# Autodesk Inventor assembly: ArmFrameWithMotorAndGears
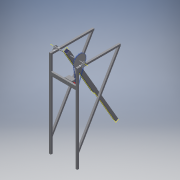
[picture p0: Inventor's stored thumbnail of the model, 180x180]
Saved by Autodesk Inventor 2018.2 (Build 222227000, 227)
## iProperties
Created: 2018-02-07
Part Number: ArmFrameWithMotorAndGears
Document SubType Name: Assembly
Designer: steele
Author: steele
## Documents named in this file (14)
- D:\snobotics\CAD-Development\robSteele\2018-FRC\Arm\ArmFrameWithMotorAndGears.iam
- D:\snobotics\CAD-Development\robSteele\2018-FRC\Arm\armFrame.ipt
- D:\snobotics\CAD-Development\robSteele\2018-FRC\Arm\hexExtrusion.ipt
- D:\snobotics\CAD-Development\robSteele\2018-FRC\Arm\ArmFrameWithMotorAndGears\Design Accelerator\Chain Drive1.iam
- D:\snobotics\CAD-Development\robSteele\2018-FRC\Arm\AM Rev 3209 Motor Mount.ipt
- D:\snobotics\CAD-Development\robSteele\2018-FRC\Arm\BaneBot220GearBox.ipt
- D:\snobotics\CAD-Development\robSteele\2018-FRC\Arm\2inSquareArmTube.ipt
- D:\snobotics\CAD-Development\robSteele\2018-FRC\Arm\1_5inSquareArmTube.ipt
- D:\snobotics\CAD-Development\robSteele\2018-FRC\Arm\30-60-supportBrace.ipt
- D:\snobotics\CAD-Development\robSteele\2018-FRC\Arm\30-60-supportBrace_MIR.ipt
- D:\snobotics\CAD-Development\robSteele\2018-FRC\Arm\ArmFrameWithMotorAndGears\Design Accelerator\Bolted Connection2.iam
- D:\snobotics\CAD-Development\robSteele\2018-FRC\Arm\ArmFrameWithMotorAndGears\Design Accelerator\Bolted Connection3.iam
- D:\snobotics\CAD-Development\robSteele\2018-FRC\Arm\ArmFrameWithMotorAndGears\Design Accelerator\Bolted Connection4.iam
- D:\snobotics\CAD-Development\robSteele\2018-FRC\Arm\ArmFrameWithMotorAndGears\Design Accelerator\Bolted Connection5.iam
## Components (14 placed, 10 different names)
1. armFrame:1 — Mate:2, Mate:3, Mate:4, Mate:5, Mate:6, Mate:7, Mate:11, Flush:2, Flush:3, Mate:15, Mate:16, Flush:4
2. hexExtrusion:1 — Flush:1, Mate:8, Mate:12, Mate:13
3. Chain Drive:1 [sub-assembly]
4. AM Rev 3209 Motor Mount:1 — Mate:2, Mate:3, Mate:4, Mate:21, Mate:22, Mate:23, Mate:24
5. AM Rev 3209 Motor Mount:2 — Mate:5, Mate:6, Mate:7, Mate:8, Mate:17, Mate:18, Mate:19, Mate:20
6. BaneBot220GearBox:1 — Mate:11, Flush:2, Flush:3
7. 2inSquareArmTube:1 — Mate:12, Mate:13, Mate:14
8. 1_5inSquareArmTube:1 — Mate:14
9. 30-60-supportBrace:1 — Mate:15, Mate:16, Flush:4
10. 30-60-supportBrace_MIR:1
11. Bolted Connection:1 [sub-assembly] — Mate:17, Mate:18
12. Bolted Connection:2 [sub-assembly] — Mate:19, Mate:20
13. Bolted Connection:3 [sub-assembly] — Mate:21, Mate:22
14. Bolted Connection:4 [sub-assembly] — Mate:23, Mate:24
## Relationships (25: Mate 21, Flush 4)
- Flush:1: hexExtrusion:1
- Mate:2: armFrame:1 ↔ AM Rev 3209 Motor Mount:1
- Mate:3: armFrame:1 ↔ AM Rev 3209 Motor Mount:1
- Mate:4 (-88.9 mm): armFrame:1 ↔ AM Rev 3209 Motor Mount:1
- Mate:5: armFrame:1 ↔ AM Rev 3209 Motor Mount:2
- Mate:6: armFrame:1 ↔ AM Rev 3209 Motor Mount:2
- Mate:7 (-88.9 mm): armFrame:1 ↔ AM Rev 3209 Motor Mount:2
- Mate:8: hexExtrusion:1 ↔ AM Rev 3209 Motor Mount:2
- Mate:11: armFrame:1 ↔ BaneBot220GearBox:1
- Flush:2 (203.2 mm): armFrame:1 ↔ BaneBot220GearBox:1
- Flush:3 (6.35 mm): armFrame:1 ↔ BaneBot220GearBox:1
- Mate:12: hexExtrusion:1 ↔ 2inSquareArmTube:1
- Mate:13: hexExtrusion:1 ↔ 2inSquareArmTube:1
- Mate:14 (-152.4 mm): 2inSquareArmTube:1 ↔ 1_5inSquareArmTube:1
- Mate:15: armFrame:1 ↔ 30-60-supportBrace:1
- Mate:16: armFrame:1 ↔ 30-60-supportBrace:1
- Flush:4: armFrame:1 ↔ 30-60-supportBrace:1
- Mate:17: AM Rev 3209 Motor Mount:2 ↔ Bolted Connection:1
- Mate:18: AM Rev 3209 Motor Mount:2 ↔ Bolted Connection:1
- Mate:19: AM Rev 3209 Motor Mount:2 ↔ Bolted Connection:2
- Mate:20: AM Rev 3209 Motor Mount:2 ↔ Bolted Connection:2
- Mate:21: AM Rev 3209 Motor Mount:1 ↔ Bolted Connection:3
- Mate:22: AM Rev 3209 Motor Mount:1 ↔ Bolted Connection:3
- Mate:23: AM Rev 3209 Motor Mount:1 ↔ Bolted Connection:4
- Mate:24: AM Rev 3209 Motor Mount:1 ↔ Bolted Connection:4
